# Autodesk Inventor assembly: cnc vertical carriage
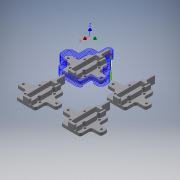
[picture p0: Inventor's stored thumbnail of the model, 180x180]
Saved by Autodesk Inventor 2016 SP1 (Build 200210100, 210)
## iProperties
Created: 2016-04-16
Part Number: cnc vertical carriage
Document SubType Name: Assembly
Designer: ubik
Author: ubik
## Documents named in this file (2)
- E:\GitHub\kossel-XXL\cnc vertical carriage.iam
- E:\GitHub\kossel-XXL\vertical carriage.ipt
## Components (4 placed, 1 different names)
1. vertical carriage:1 — Flush:1, Flush:2, Flush:3, Flush:4, Mate:1, Flush:6
2. vertical carriage:2 — Flush:1, Flush:4, Mate:1, Mate:3
3. vertical carriage:3 — Flush:2, Flush:5, Mate:2, Mate:3, Flush:6
4. vertical carriage:4 — Flush:3, Flush:5, Mate:2
## Relationships (9: Flush 6, Mate 3)
- Flush:1: vertical carriage:1 ↔ vertical carriage:2
- Flush:2: vertical carriage:1 ↔ vertical carriage:3
- Flush:3: vertical carriage:1 ↔ vertical carriage:4
- Flush:4: vertical carriage:1 ↔ vertical carriage:2
- Flush:5: vertical carriage:3 ↔ vertical carriage:4
- Mate:1 (8 mm): vertical carriage:1 ↔ vertical carriage:2
- Mate:2 (8 mm): vertical carriage:3 ↔ vertical carriage:4
- Mate:3 (8 mm): vertical carriage:2 ↔ vertical carriage:3
- Flush:6: vertical carriage:1 ↔ vertical carriage:3
